# Autodesk Inventor assembly: Projector_PCB
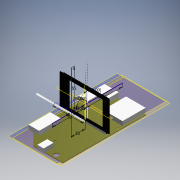
[picture p0: Inventor's stored thumbnail of the model, 180x180]
Saved by Autodesk Inventor 2016 (Build 200138000, 138)
## iProperties
Created: 2016-11-13
Part Number: Projector_PCB
Material: Generisch
Document SubType Name: Assembly
Designer: Bene
Author: Bene
## Documents named in this file (5)
- C:\Users\Bene\Dropbox\Dokumente\OpticalDesign\Beamerscope\Inventor\Beamerscope_r4\Projector_PCB.iam
- C:\Users\Bene\Dropbox\Dokumente\OpticalDesign\Beamerscope\Inventor\Beamerscope_r4\01_PCBoard.ipt
- C:\Users\Bene\Dropbox\Dokumente\OpticalDesign\Beamerscope\Inventor\Beamerscope_r4\02_Anschluss.ipt
- C:\Users\Bene\Dropbox\Dokumente\OpticalDesign\Beamerscope\Inventor\Beamerscope_r4\03_LCD_Frame.ipt
- C:\Users\Bene\Dropbox\Dokumente\OpticalDesign\Beamerscope\Inventor\Beamerscope_r4\04_Mirror.ipt
## Components (4 placed, 4 different names)
1. 01_PCBoard:1
2. 02_Anschluss:1
3. 03_LCD_Frame:1
4. 04_Mirror:1
## Relationships (6: Flush 6)
- [Flush]: 01_PCBoard:1 ↔ 02_Anschluss:1
- [Flush]: 01_PCBoard:1 ↔ 02_Anschluss:1
- [Flush] (4 mm): 01_PCBoard:1 ↔ 03_LCD_Frame:1
- [Flush] (-2 mm): 01_PCBoard:1 ↔ 03_LCD_Frame:1
- [Flush] (63 mm): 01_PCBoard:1 ↔ 03_LCD_Frame:1
- [Flush]: 01_PCBoard:1 ↔ 02_Anschluss:1
## Named parameters: d0_d3 = -2 mm, d1_d4 = 63 mm, d2_d5 = 0 mm
